# Autodesk Inventor assembly: 6P Sprocket
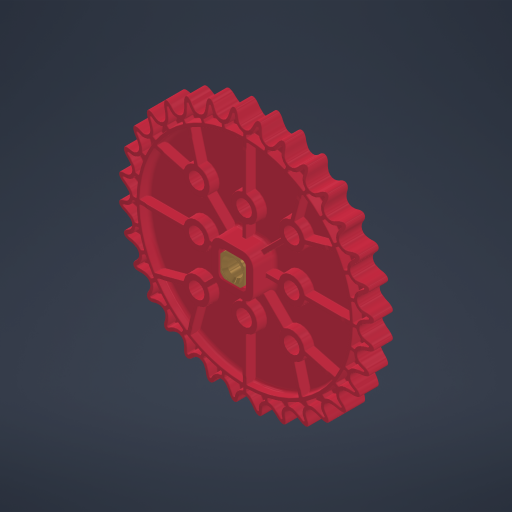
[picture p0: Inventor's stored thumbnail of the model, 512x512]
Saved by Autodesk Inventor 2023.2 (Build 272271000, 271)
## iProperties
Created: 2022-08-02
Part Number: 6P Sprocket
Document SubType Name: Assembly
Designer: ylu12
Author: ylu12
## Documents named in this file (4)
- D:\CAD\Parts\standard\Motion\Chain\6P Sprocket\6P 32T Sprocket, Circle.iam
- D:\CAD\Parts\standard\Motion\Adapters\HS Shaft Adapter Circle.ipt
- D:\CAD\Parts\standard\Motion\Chain\Reference parts\6P 32T Sprocket.ipt
- D:\CAD\Parts\standard\Motion\Chain\6P Sprocket.iam
## Components (2 placed, 2 different names)
1. Circle — Flush:1, Mate:1, Mate:3
2. 32T — Flush:6, Mate:11, Mate:12
## Relationships (6: Mate 4, Flush 2)
- Flush:1 (6.35 mm): Circle
- Mate:1: Circle
- Mate:3: Circle
- Flush:6: 32T
- Mate:11: 32T
- Mate:12: 32T
